# Autodesk Inventor assembly: 2024-000
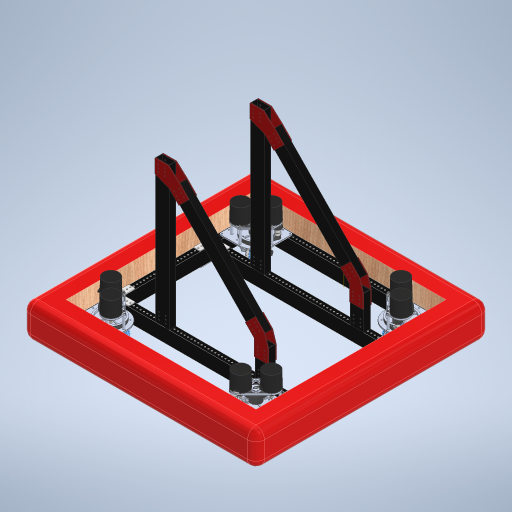
[picture p0: Inventor's stored thumbnail of the model, 512x512]
Saved by Autodesk Inventor 2024.2 (Build 282272000, 272)
## iProperties
Created: 2024-01-07
Part Number: 2024-000
Document SubType Name: Assembly
Designer: rohan
Author: rohan
## Documents named in this file (3)
- C:\Users\rohan\OneDrive - Hillsborough County Public Schools\Robotics\FIRST-Robotics-Competition\Crescendo\Minotaur-Crescendo-Robot\2024-000.iam
- C:\Users\rohan\OneDrive - Hillsborough County Public Schools\Robotics\FIRST-Robotics-Competition\Crescendo\Minotaur-Crescendo-Robot\Swerve-Drivetrain-2.iam
- C:\Users\rohan\OneDrive - Hillsborough County Public Schools\Robotics\FIRST-Robotics-Competition\Crescendo\Minotaur-Crescendo-Robot\Structure\Superstructure\2024-210-Superstructure.iam
## Components (2 placed, 2 different names)
1. Swerve-Drivetrain-2:1 [sub-assembly] — Flush:1, Mate:1
2. 2024-210-Superstructure:1 [sub-assembly] — Flush:1, Mate:1
## Relationships (2: Flush 1, Mate 1)
- Flush:1: Swerve-Drivetrain-2:1 ↔ 2024-210-Superstructure:1
- Mate:1: Swerve-Drivetrain-2:1 ↔ 2024-210-Superstructure:1
